# Autodesk Inventor assembly: Upper Stage
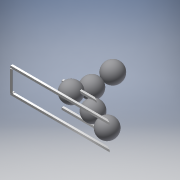
[picture p0: Inventor's stored thumbnail of the model, 180x180]
Saved by Autodesk Inventor 2019.4 (Build 234330000, 330)
## iProperties
Created: 2020-01-18
Part Number: Upper Stage
Document SubType Name: Assembly
Designer: Mark
Mass: 1292.77 g
Surface Area: 4691.82 cm^2
Volume: 478.802 cm^3
Density: 2.7 g/cm^3
Author: Mark
## Documents named in this file (5)
- C:\Users\Mark\Desktop\7738 Helion Engineering\7738-2020\Upper Stage\Upper Stage.iam
- C:\Users\Mark\Desktop\7738 Helion Engineering\7738-2020\Upper Stage\Main Extrusions.ipt
- C:\Users\Mark\Desktop\7738 Helion Engineering\7738-2020\Upper Stage\Back Support Piece.ipt
- C:\Users\Mark\Desktop\7738 Helion Engineering\7738-2020\Upper Stage\Secondary Extrusions.ipt
- C:\Users\Mark\Desktop\7738 Helion Engineering\7738-2020\Power Cell.ipt
## Components (10 placed, 4 different names)
1. Main Extrusions:1 — Mate:1, Flush:1, Flush:2, Flush:8
2. Main Extrusions:2 — Mate:1, Flush:1, Flush:2, Flush:3, Flush:4, Mate:2, Flush:5, Flush:7, Mate:3
3. Back Support Piece:1 — Flush:3, Flush:4, Mate:2
4. Secondary Extrusions:1 — Flush:5, Flush:7, Flush:9, Mate:3, Flush:10
5. Secondary Extrusions:2 — Flush:8, Flush:9, Flush:10
6. Power Cell:1
7. Power Cell:2
8. Power Cell:3
9. Power Cell:4
10. Power Cell:5
## Relationships (12: Flush 9, Mate 3)
- Mate:1 (200 mm): Main Extrusions:1 ↔ Main Extrusions:2
- Flush:1: Main Extrusions:1 ↔ Main Extrusions:2
- Flush:2: Main Extrusions:1 ↔ Main Extrusions:2
- Flush:3: Main Extrusions:2 ↔ Back Support Piece:1
- Flush:4: Main Extrusions:2 ↔ Back Support Piece:1
- Mate:2: Main Extrusions:2 ↔ Back Support Piece:1
- Flush:5: Main Extrusions:2 ↔ Secondary Extrusions:1
- Flush:7: Main Extrusions:2 ↔ Secondary Extrusions:1
- Flush:8: Main Extrusions:1 ↔ Secondary Extrusions:2
- Flush:9: Secondary Extrusions:1 ↔ Secondary Extrusions:2
- Mate:3 (100 mm): Main Extrusions:2 ↔ Secondary Extrusions:1
- Flush:10: Secondary Extrusions:1 ↔ Secondary Extrusions:2
